# Autodesk Inventor assembly: Leg-40x
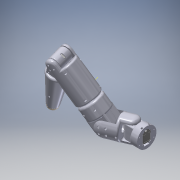
[picture p0: Inventor's stored thumbnail of the model, 180x180]
Saved by Autodesk Inventor 2018 (Build 220112000, 112)
## iProperties
Created: 2017-08-15
Part Number: Leg-40x
Material: Generisch
Document SubType Name: Assembly
Designer: JochenAlt
Author: JochenAlt
## Documents named in this file (8)
- D:\Projects\Manfred\design\cad\Inventor\Leg-40x.iam
- D:\Projects\Manfred\design\cad\Inventor\HipJoint-40x.ipt
- D:\Projects\Manfred\design\cad\Inventor\Thigh-40x.iam
- D:\Projects\Manfred\design\cad\Inventor\Herkulex DRS-010x\HerkuleX DRS-0101.iam
- D:\Projects\Manfred\design\cad\Inventor\Hip-40x.ipt
- D:\Projects\Manfred\design\cad\Inventor\Rillenkugellager 11x7x3 inafag smr117.ipt
- D:\Projects\Manfred\design\cad\Inventor\Servobackaxis.ipt
- D:\Projects\Manfred\design\cad\Inventor\Foot-40x.iam
## Components (8 placed, 7 different names)
1. HipJoint-40x:1 — Passend:23, Passend:24, Passend:29, Passend:30, Passend:34, Passend:35, Passend:36, Passend:37, Passend:38, Passend:41
2. Thigh-40x:1 [sub-assembly] — Passend:23, Passend:24, Passend:36, Passend:37, Passend:38, Passend:39, Passend:40, Passend:42, Passend:43
3. HerkuleX DRS-0101:1 [sub-assembly] — Passend:3, Passend:4, Passend:5, Passend:27
4. Hip-40x:1 — Passend:3, Passend:4, Passend:5, Passend:33
5. Rillenkugellager 11x7x3 inafag smr117:1 — Passend:27, Passend:31, Passend:32, Passend:33
6. Servobackaxis:1 — Passend:29, Passend:30, Passend:31, Passend:32, Passend:34, Passend:35
7. Rillenkugellager 11x7x3 inafag smr117:2 — Passend:39, Passend:40, Passend:41
8. Foot-40x:1 [sub-assembly] — Passend:42, Passend:43
## Relationships (21: Mate 21)
- Passend:3 [Mate]: HerkuleX DRS-0101:1 ↔ Hip-40x:1
- Passend:4 [Mate]: HerkuleX DRS-0101:1 ↔ Hip-40x:1
- Passend:5 [Mate]: HerkuleX DRS-0101:1 ↔ Hip-40x:1
- Passend:23 [Mate]: HipJoint-40x:1 ↔ Thigh-40x:1
- Passend:24 [Mate]: HipJoint-40x:1 ↔ Thigh-40x:1
- Passend:27 [Mate]: HerkuleX DRS-0101:1 ↔ Rillenkugellager 11x7x3 inafag smr117:1
- Passend:29 [Mate]: HipJoint-40x:1 ↔ Servobackaxis:1
- Passend:30 [Mate]: HipJoint-40x:1 ↔ Servobackaxis:1
- Passend:31 [Mate]: Rillenkugellager 11x7x3 inafag smr117:1 ↔ Servobackaxis:1
- Passend:32 [Mate]: Rillenkugellager 11x7x3 inafag smr117:1 ↔ Servobackaxis:1
- Passend:33 [Mate]: Hip-40x:1 ↔ Rillenkugellager 11x7x3 inafag smr117:1
- Passend:34 [Mate]: HipJoint-40x:1 ↔ Servobackaxis:1
- Passend:35 [Mate]: HipJoint-40x:1 ↔ Servobackaxis:1
- Passend:36 [Mate]: HipJoint-40x:1 ↔ Thigh-40x:1
- Passend:37 [Mate]: HipJoint-40x:1 ↔ Thigh-40x:1
- Passend:38 [Mate]: HipJoint-40x:1 ↔ Thigh-40x:1
- Passend:39 [Mate]: Thigh-40x:1 ↔ Rillenkugellager 11x7x3 inafag smr117:2
- Passend:40 [Mate]: Thigh-40x:1 ↔ Rillenkugellager 11x7x3 inafag smr117:2
- Passend:41 [Mate]: HipJoint-40x:1 ↔ Rillenkugellager 11x7x3 inafag smr117:2
- Passend:42 [Mate]: Thigh-40x:1 ↔ Foot-40x:1
- Passend:43 [Mate]: Thigh-40x:1 ↔ Foot-40x:1
